# Autodesk Inventor assembly: Laser_alignment
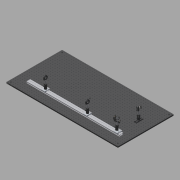
[picture p0: Inventor's stored thumbnail of the model, 180x180]
Saved by Autodesk Inventor 2018 (Build 220112000, 112)
## iProperties
Created: 2018-09-17
Part Number: Laser_alignment
Document SubType Name: Assembly
Designer: Robert Campbell
Author: Robert Campbell
## Documents named in this file (6)
- \\Mac\Home\Dropbox\home\work\Microscopes\SWC_Optics_course_2018\Laser_alignment.iam
- \\Mac\Home\Downloads\LaserAlignment\MB60120_M-Solidworks.ipt
- \\Mac\Home\Downloads\LaserAlignment\XT66DP-1000-Solidworks.ipt
- \\Mac\Home\Downloads\LaserAlignment\Iris_On_Carriage.iam
- \\Mac\Home\Downloads\LaserAlignment\Mirror_on_carriage.iam
- \\Mac\Home\Downloads\LaserAlignment\first_mirror.iam
## Components (6 placed, 5 different names)
1. MB60120_M-Solidworks:1 — Mate:1, Mate:21, Angle:4
2. XT66DP-1000-Solidworks:1 — Mate:1, Angle:1, Mate:16, Mate:17, Angle:2, Mate:18, Mate:19, Angle:3, Mate:20
3. Iris_On_Carriage:1 [sub-assembly] — Angle:2, Mate:18, Mate:19
4. Iris_On_Carriage:2 [sub-assembly] — Angle:1, Mate:16, Mate:17
5. Mirror_on_carriage:1 [sub-assembly] — Angle:3, Mate:20
6. first_mirror:1 [sub-assembly] — Mate:21, Angle:4
## Relationships (11: Mate 7, Angle 4)
- Mate:1: MB60120_M-Solidworks:1 ↔ XT66DP-1000-Solidworks:1
- Angle:1 (0 deg): XT66DP-1000-Solidworks:1 ↔ Iris_On_Carriage:2
- Mate:16: XT66DP-1000-Solidworks:1 ↔ Iris_On_Carriage:2
- Mate:17: XT66DP-1000-Solidworks:1 ↔ Iris_On_Carriage:2
- Angle:2 (0 deg): XT66DP-1000-Solidworks:1 ↔ Iris_On_Carriage:1
- Mate:18: XT66DP-1000-Solidworks:1 ↔ Iris_On_Carriage:1
- Mate:19: XT66DP-1000-Solidworks:1 ↔ Iris_On_Carriage:1
- Angle:3 (0 deg): XT66DP-1000-Solidworks:1 ↔ Mirror_on_carriage:1
- Mate:20: XT66DP-1000-Solidworks:1 ↔ Mirror_on_carriage:1
- Mate:21: MB60120_M-Solidworks:1 ↔ first_mirror:1
- Angle:4 (0 deg): MB60120_M-Solidworks:1 ↔ first_mirror:1
